# Autodesk Inventor assembly: Assembly1
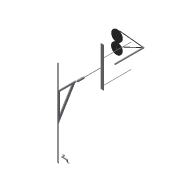
[picture p0: Inventor's stored thumbnail of the model, 180x180]
Saved by Autodesk Inventor 2017 (Build 210142000, 142)
## iProperties
Created: 2019-07-23
Part Number: Assembly1
Document SubType Name: Assembly
Designer: Admin
Author: Admin
## Documents named in this file (10)
- E:\PK\8 mechanism\Prototype 1\Table move\Assembly1.iam
- E:\PK\8 mechanism\Prototype 1\Table move\Part21.ipt
- E:\PK\8 mechanism\Prototype 1\Table move\Part2.ipt
- E:\PK\8 mechanism\Prototype 1\Table move\Part7.ipt
- E:\PK\8 mechanism\Prototype 1\Table move\Part1.ipt
- E:\PK\8 mechanism\Prototype 1\Table move\Part12.ipt
- E:\PK\8 mechanism\Prototype 1\Part1.ipt
- E:\PK\8 mechanism\Prototype 1\Part2.ipt
- E:\PK\8 mechanism\Prototype 1\Part3.ipt
- E:\PK\8 mechanism\Prototype 1\Table move\Part122.ipt
## Components (13 placed, 7 different names)
1. Part21:1 — Angle:2, Slider:1, Transitional:2, Mate:6
2. Part2:1 — Angle:1, Tangent:1, Rotation/Translation:1, Slider:1, Transitional:2, Mate:4
3. Part7:1 — Angle:1, Tangent:1, Mate:3, Transitional:1, Mate:4, Angle:4, Angle:5
4. Part1:1 — Mate:3, Transitional:1
5. Part12:1 — Angle:2, Rotation/Translation:1, Rotational:1, Rotation:2
6. Part12:2 — Rotational:1
7. Part1:2 — Tangent:2, Angle:5, Insert:1, Insert:3, Flush:1, Rotation:1, Rotation:2, Mate:6
8. Part1:3 — Angle:4, Tangent:2, Insert:2, Insert:4, Flush:1, Rotation:1
9. Part2:2 — Insert:1
10. Part2:3 — Insert:2
11. Part3:1 — Insert:3, Mate:5
12. Part3:2 — Insert:4, Mate:5, Insert:5
13. Part122:1 — Insert:5
## Relationships (23: Insert 5, Angle 4, Mate 4, Tangent 2, Transitional 2, RelateRotation 2, RelateRotateTranslate 1, RevoluteJoint 1, TranslationJoint 1, Flush 1)
- Angle:1 (0 deg): Part2:1 ↔ Part7:1
- Tangent:1: Part2:1 ↔ Part7:1
- Mate:3: Part7:1 ↔ Part1:1
- Angle:2 (0 deg): Part21:1 ↔ Part12:1
- Rotation/Translation:1 [RelateRotateTranslate] (50 mm): Part2:1 ↔ Part12:1
- Rotational:1 [RevoluteJoint]: Part12:1 ↔ Part12:2
- Slider:1 [TranslationJoint]: Part21:1 ↔ Part2:1
- Transitional:1: Part7:1 ↔ Part1:1
- Transitional:2: Part21:1 ↔ Part2:1
- Mate:4 (0.422 mm): Part2:1 ↔ Part7:1
- Angle:4 (180 deg): Part7:1 ↔ Part1:3
- Tangent:2: Part1:2 ↔ Part1:3
- Angle:5 (180 deg): Part7:1 ↔ Part1:2
- Insert:1: Part1:2 ↔ Part2:2
- Insert:2: Part1:3 ↔ Part2:3
- Insert:3: Part1:2 ↔ Part3:1
- Insert:4: Part1:3 ↔ Part3:2
- Flush:1: Part1:2 ↔ Part1:3
- Mate:5: Part3:1 ↔ Part3:2
- Rotation:1 [RelateRotation] (1 ul): Part1:2 ↔ Part1:3
- Rotation:2 [RelateRotation] (1 ul): Part12:1 ↔ Part1:2
- Mate:6 (1665.291 mm): Part21:1 ↔ Part1:2
- Insert:5: Part3:2 ↔ Part122:1
